# Autodesk Inventor assembly: WristAssembly
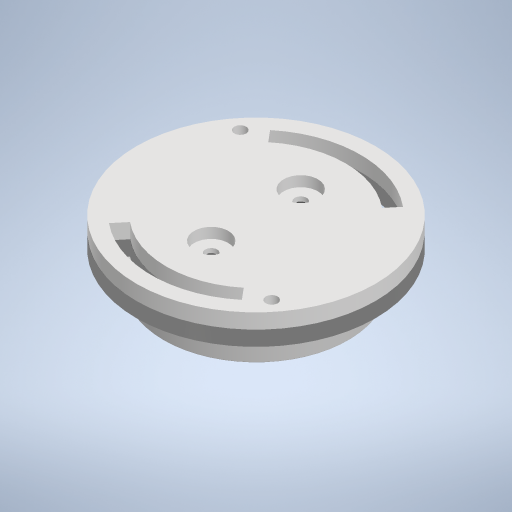
[picture p0: Inventor's stored thumbnail of the model, 512x512]
Saved by Autodesk Inventor 2023 (Build 270158000, 158)
## iProperties
Created: 2023-04-09
Part Number: WristAssembly
Document SubType Name: Assembly
Designer: adity
Author: adity
## Documents named in this file (5)
- C:\Users\1senadi\Downloads\WristAssembly.iam
- C:\Users\1senadi\Downloads\Wrist-Bearing Attachment.ipt
- C:\Users\1senadi\Downloads\Wrist_Arm.ipt
- C:\Users\1senadi\Downloads\SKF_CAD_MODEL_SKF_W 61710\AIS2023\SKF_W 61710.iam
- C:\Users\1senadi\Downloads\Wrist_Coupling.ipt
## Components (4 placed, 4 different names)
1. Wrist_Arm:1 — Insert:1, Insert:3
2. Wrist-Bearing Attachment:2 — Insert:1, Insert:2
3. SKF_W 61710:1 [sub-assembly] — Insert:2
4. Wrist_Coupling:1 — Insert:3
## Relationships (3: Insert 3)
- Insert:1: Wrist_Arm:1 ↔ Wrist-Bearing Attachment:2
- Insert:2: Wrist-Bearing Attachment:2 ↔ SKF_W 61710:1
- Insert:3: Wrist_Arm:1 ↔ Wrist_Coupling:1
